# Autodesk Inventor assembly: Bevel Gear Assembly
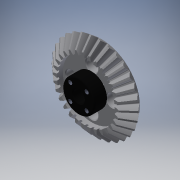
[picture p0: Inventor's stored thumbnail of the model, 180x180]
Saved by Autodesk Inventor 2016 (Build 200138000, 138)
## iProperties
Created: 2015-10-16
Part Number: Bevel Gear Assembly
Document SubType Name: Assembly
Designer: hppeng
Author: hppeng
## Documents named in this file (3)
- C:\Users\hppeng\Desktop\Jing-Chen Stuffs\FTC\Bionic-Hybrids\CAD\General\Modified Parts\Bevel Gear Assembly.iam
- C:\Users\hppeng\Desktop\Jing-Chen Stuffs\FTC\Bionic-Hybrids\Stock\Bevel Gear - 738007.ipt
- C:\Users\hppeng\Desktop\Jing-Chen Stuffs\FTC\Bionic-Hybrids\Stock\Bevel Gear Spacer - 738008.ipt
## Components (2 placed, 2 different names)
1. Bevel Gear - 738007:1 — Mate:1, Mate:2, Mate:3
2. Bevel Gear Spacer - 738008:1 — Mate:1, Mate:2, Mate:3
## Relationships (3: Mate 3)
- Mate:1: Bevel Gear - 738007:1 ↔ Bevel Gear Spacer - 738008:1
- Mate:2: Bevel Gear - 738007:1 ↔ Bevel Gear Spacer - 738008:1
- Mate:3: Bevel Gear - 738007:1 ↔ Bevel Gear Spacer - 738008:1
